# Autodesk Inventor assembly: Catapult Launcher
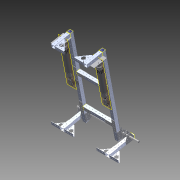
[picture p0: Inventor's stored thumbnail of the model, 180x180]
Saved by Autodesk Inventor 2014 (Build 180170000, 170)
## iProperties
Created: 2014-01-17
Part Number: Catapult Launcher
Document SubType Name: Assembly
Designer: Andrew Toennies
Mass: 1552.27 g
Surface Area: 5150.08 cm^2
Volume: 383.1 cm^3
Density: 4.05187 g/cm^3
Author: Andrew Toennies
## Documents named in this file (14)
- C:\Users\Andrew Toennies\Documents\GitHub\2014buildCAD\New Shooter\Catapult Launcher.iam
- C:\Users\Andrew Toennies\Documents\GitHub\2014buildCAD\New Shooter\Vex Pro 1x1 rectangular tubing 7 in length.ipt
- C:\Users\Andrew Toennies\Documents\GitHub\2014buildCAD\New Shooter\Vex Pro Side Bearing Gusset.ipt
- C:\Users\Andrew Toennies\Documents\GitHub\2014buildCAD\New Shooter\Vex Pro Corner Gusset.ipt
- C:\Users\Andrew Toennies\Documents\GitHub\2014buildCAD\New Shooter\Bearing ID 0.500 Hex OD 1.125.ipt
- C:\Users\Andrew Toennies\Documents\GitHub\2014buildCAD\New Shooter\Shaft (Steel 0.500 Hex).ipt
- C:\Users\Andrew Toennies\Documents\GitHub\2014buildCAD\New Shooter\Vex Pro 1x1 rectangular tubing 27 in length.ipt
- C:\Users\Andrew Toennies\Documents\GitHub\2014buildCAD\New Shooter\Vex Pro 1x1 rectangular tubing 3 in length.ipt
- C:\Users\Andrew Toennies\Documents\GitHub\2014buildCAD\New Shooter\Vex Pro 1x1 rectangular tubing 11 in length.ipt
- C:\Users\Andrew Toennies\Documents\GitHub\2014buildCAD\New Shooter\Vex Pro T gusset.ipt
- C:\Users\Andrew Toennies\Documents\GitHub\2014buildCAD\New Shooter\1.5 in bore 6 in stroke cylinder - BIMBA\176-DP(D-229)(F,D-231-1).iam
- C:\Users\Andrew Toennies\Documents\GitHub\2014buildCAD\New Shooter\Aluminum Plate (0.125).ipt
- C:\Users\Andrew Toennies\Documents\GitHub\2014buildCAD\New Shooter\1.5 in bore 6 in stroke cylinder - BIMBA\D-14826.ipt
- C:\Users\Andrew Toennies\Documents\GitHub\2014buildCAD\New Shooter\1.5 in bore 6 in stroke cylinder - BIMBA\D-9969.ipt
## Components (45 placed, 13 different names)
1. Shaft (Steel 0.500 Hex):1 — Mate:34, Mate:35, Flush:25
2. Vex Pro 1x1 rectangular tubing 3 in length:1 — Flush:13, Mate:118, Mate:119, Mate:120, Mate:123, Flush:19, Mate:160, Mate:212
3. Vex Pro 1x1 rectangular tubing 3 in length:2 — Mate:121, Flush:14, Mate:122, Flush:19, Mate:159
4. Vex Pro 1x1 rectangular tubing 11 in length:1 — Mate:140, Mate:141, Mate:142, Mate:143, Mate:146, Mate:147, Mate:148, Mate:149, Mate:191, Mate:193, Mate:194, Mate:196, Mate:197
5. Vex Pro 1x1 rectangular tubing 11 in length:2 — Mate:127, Mate:128, Mate:129, Mate:131, Mate:135, Mate:136, Mate:137, Mate:185
6. Vex Pro T gusset:1 — Mate:140, Mate:141, Mate:142, Mate:201, Mate:202
7. Vex Pro T gusset:2 — Mate:143, Mate:193, Mate:194
8. Vex Pro T gusset:3 — Mate:127, Mate:128, Mate:129, Mate:203, Mate:204, Mate:205
9. Vex Pro T gusset:4 — Mate:146, Mate:147, Mate:148
10. Vex Pro T gusset:5 — Mate:135, Mate:136, Mate:185
11. Vex Pro T gusset:6 — Mate:137, Mate:210, Mate:211
12. Vex Pro T gusset:7 — Mate:149, Mate:196, Mate:197
13. Vex Pro T gusset:8 — Mate:131, Mate:187, Mate:192
14. Aluminum Plate (0.125):1 — Mate:153, Mate:154, Mate:155, Mate:159, Flush:24
15. Aluminum Plate (0.125):2 — Mate:156, Mate:160, Mate:167, Mate:168, Flush:24
16. D-14826:1 — Mate:164, Mate:169, Mate:170, Mate:177, Mate:178
17. D-9969:1 — Mate:164, Mate:165, Mate:166, Mate:198, Mate:199, Mate:200
18. Vex Pro 1x1 rectangular tubing 27 in length:3 — Mate:198, Mate:199, Mate:200, Mate:201, Mate:202, Mate:203, Mate:204, Mate:205, Mate:206, Mate:207, Mate:208, Mate:209, Mate:213
19. Vex Pro 1x1 rectangular tubing 7 in length:1 — Flush:1, Flush:2, Mate:8, Mate:11, Mate:20, Mate:21, Mate:22, Mate:23, Mate:24, Mate:25, Mate:114, Mate:115, Mate:116, Mate:117, Mate:195
20. Vex Pro 1x1 rectangular tubing 7 in length:2 — Flush:1, Flush:2, Mate:3, Mate:5, Mate:14, Mate:15, Mate:16, Mate:17, Mate:18, Mate:19, Mate:110, Mate:111, Mate:112, Mate:113, Mate:123, Mate:188, Mate:195, Flush:25
21. Vex Pro Side Bearing Gusset:1 — Mate:3, Mate:26, Mate:27, Mate:110, Mate:111
22. Vex Pro Side Bearing Gusset:2 — Mate:5, Mate:28, Mate:29, Mate:112, Mate:113
23. Vex Pro Side Bearing Gusset:3 — Mate:11, Mate:32, Mate:33, Mate:116, Mate:117
24. Vex Pro Side Bearing Gusset:4 — Mate:8, Mate:30, Mate:31, Mate:114, Mate:115
25. Vex Pro Corner Gusset:1 — Mate:17, Mate:18, Mate:19, Flush:18
26. Vex Pro Corner Gusset:2 — Mate:14, Mate:15, Mate:16
27. Vex Pro Corner Gusset:3 — Mate:20, Mate:21, Mate:22
28. Vex Pro Corner Gusset:4 — Mate:23, Mate:24, Mate:25
29. Bearing ID 0.500 Hex OD 1.125:1 — Mate:28, Mate:29, Flush:3, Flush:5
30. Bearing ID 0.500 Hex OD 1.125:2 — Mate:26, Mate:27, Flush:3, Mate:34, Mate:35, Mate:44
31. Bearing ID 0.500 Hex OD 1.125:3 — Mate:30, Mate:31, Flush:4
32. Bearing ID 0.500 Hex OD 1.125:4 — Mate:32, Mate:33, Flush:4, Flush:5, Mate:69
33. Vex Pro Side Bearing Gusset:5 — Mate:57, Mate:58, Mate:180, Mate:181, Mate:189
34. Vex Pro Side Bearing Gusset:6 — Mate:55, Mate:56, Mate:208, Mate:209, Mate:213
35. Vex Pro Side Bearing Gusset:7 — Mate:51, Mate:52, Mate:206, Mate:207
36. Vex Pro Side Bearing Gusset:8 — Mate:44, Mate:53, Mate:54, Mate:179, Mate:182
37. Vex Pro 1x1 rectangular tubing 27 in length:2 — Mate:177, Mate:178, Mate:179, Mate:180, Mate:181, Mate:182, Mate:187, Mate:188, Mate:189, Mate:191, Mate:192, Mate:210, Mate:211, Mate:212
38. Bearing ID 0.500 Hex OD 1.125:5 — Mate:57, Mate:58, Mate:80
39. Bearing ID 0.500 Hex OD 1.125:6 — Mate:53, Mate:54, Mate:80
40. Bearing ID 0.500 Hex OD 1.125:7 — Mate:51, Mate:52, Mate:68, Mate:69
41. Bearing ID 0.500 Hex OD 1.125:8 — Mate:55, Mate:56, Mate:68
42. Vex Pro Corner Gusset:8 — Flush:13, Mate:118, Mate:119, Mate:120, Flush:17, Flush:18
43. Vex Pro Corner Gusset:6 — Mate:121, Flush:14, Mate:122, Flush:17
44. 176-DP(D-229)(F,D-231-1):1 [sub-assembly] — Mate:153, Mate:154, Mate:155, Mate:165, Mate:166, Mate:171
45. 176-DP(D-229)(F,D-231-1):2 [sub-assembly] — Mate:156, Mate:167, Mate:168, Mate:169, Mate:170, Mate:171
## Relationships (126: Mate 114, Flush 12)
- Flush:1: Vex Pro 1x1 rectangular tubing 7 in length:1 ↔ Vex Pro 1x1 rectangular tubing 7 in length:2
- Flush:2: Vex Pro 1x1 rectangular tubing 7 in length:1 ↔ Vex Pro 1x1 rectangular tubing 7 in length:2
- Mate:3: Vex Pro 1x1 rectangular tubing 7 in length:2 ↔ Vex Pro Side Bearing Gusset:1
- Mate:5: Vex Pro 1x1 rectangular tubing 7 in length:2 ↔ Vex Pro Side Bearing Gusset:2
- Mate:8: Vex Pro 1x1 rectangular tubing 7 in length:1 ↔ Vex Pro Side Bearing Gusset:4
- Mate:11: Vex Pro 1x1 rectangular tubing 7 in length:1 ↔ Vex Pro Side Bearing Gusset:3
- Mate:14: Vex Pro 1x1 rectangular tubing 7 in length:2 ↔ Vex Pro Corner Gusset:2
- Mate:15: Vex Pro 1x1 rectangular tubing 7 in length:2 ↔ Vex Pro Corner Gusset:2
- Mate:16: Vex Pro 1x1 rectangular tubing 7 in length:2 ↔ Vex Pro Corner Gusset:2
- Mate:17: Vex Pro 1x1 rectangular tubing 7 in length:2 ↔ Vex Pro Corner Gusset:1
- Mate:18: Vex Pro 1x1 rectangular tubing 7 in length:2 ↔ Vex Pro Corner Gusset:1
- Mate:19: Vex Pro 1x1 rectangular tubing 7 in length:2 ↔ Vex Pro Corner Gusset:1
- Mate:20: Vex Pro 1x1 rectangular tubing 7 in length:1 ↔ Vex Pro Corner Gusset:3
- Mate:21: Vex Pro 1x1 rectangular tubing 7 in length:1 ↔ Vex Pro Corner Gusset:3
- Mate:22: Vex Pro 1x1 rectangular tubing 7 in length:1 ↔ Vex Pro Corner Gusset:3
- Mate:23: Vex Pro 1x1 rectangular tubing 7 in length:1 ↔ Vex Pro Corner Gusset:4
- Mate:24: Vex Pro 1x1 rectangular tubing 7 in length:1 ↔ Vex Pro Corner Gusset:4
- Mate:25: Vex Pro 1x1 rectangular tubing 7 in length:1 ↔ Vex Pro Corner Gusset:4
- Mate:26: Vex Pro Side Bearing Gusset:1 ↔ Bearing ID 0.500 Hex OD 1.125:2
- Mate:27: Vex Pro Side Bearing Gusset:1 ↔ Bearing ID 0.500 Hex OD 1.125:2
- Mate:28: Vex Pro Side Bearing Gusset:2 ↔ Bearing ID 0.500 Hex OD 1.125:1
- Mate:29: Vex Pro Side Bearing Gusset:2 ↔ Bearing ID 0.500 Hex OD 1.125:1
- Flush:3: Bearing ID 0.500 Hex OD 1.125:1 ↔ Bearing ID 0.500 Hex OD 1.125:2
- Mate:30: Vex Pro Side Bearing Gusset:4 ↔ Bearing ID 0.500 Hex OD 1.125:3
- Mate:31: Vex Pro Side Bearing Gusset:4 ↔ Bearing ID 0.500 Hex OD 1.125:3
- Mate:32: Vex Pro Side Bearing Gusset:3 ↔ Bearing ID 0.500 Hex OD 1.125:4
- Mate:33: Vex Pro Side Bearing Gusset:3 ↔ Bearing ID 0.500 Hex OD 1.125:4
- Flush:4: Bearing ID 0.500 Hex OD 1.125:3 ↔ Bearing ID 0.500 Hex OD 1.125:4
- Flush:5: Bearing ID 0.500 Hex OD 1.125:1 ↔ Bearing ID 0.500 Hex OD 1.125:4
- Mate:34: Shaft (Steel 0.500 Hex):1 ↔ Bearing ID 0.500 Hex OD 1.125:2
- Mate:35: Shaft (Steel 0.500 Hex):1 ↔ Bearing ID 0.500 Hex OD 1.125:2
- Mate:44: Bearing ID 0.500 Hex OD 1.125:2 ↔ Vex Pro Side Bearing Gusset:8
- Mate:51: Vex Pro Side Bearing Gusset:7 ↔ Bearing ID 0.500 Hex OD 1.125:7
- Mate:52: Vex Pro Side Bearing Gusset:7 ↔ Bearing ID 0.500 Hex OD 1.125:7
- Mate:53: Vex Pro Side Bearing Gusset:8 ↔ Bearing ID 0.500 Hex OD 1.125:6
- Mate:54: Vex Pro Side Bearing Gusset:8 ↔ Bearing ID 0.500 Hex OD 1.125:6
- Mate:55: Vex Pro Side Bearing Gusset:6 ↔ Bearing ID 0.500 Hex OD 1.125:8
- Mate:56: Vex Pro Side Bearing Gusset:6 ↔ Bearing ID 0.500 Hex OD 1.125:8
- Mate:57: Vex Pro Side Bearing Gusset:5 ↔ Bearing ID 0.500 Hex OD 1.125:5
- Mate:58: Vex Pro Side Bearing Gusset:5 ↔ Bearing ID 0.500 Hex OD 1.125:5
- Mate:68: Bearing ID 0.500 Hex OD 1.125:7 ↔ Bearing ID 0.500 Hex OD 1.125:8
- Mate:69: Bearing ID 0.500 Hex OD 1.125:4 ↔ Bearing ID 0.500 Hex OD 1.125:7
- Mate:80: Bearing ID 0.500 Hex OD 1.125:5 ↔ Bearing ID 0.500 Hex OD 1.125:6
- Mate:110: Vex Pro 1x1 rectangular tubing 7 in length:2 ↔ Vex Pro Side Bearing Gusset:1
- Mate:111: Vex Pro 1x1 rectangular tubing 7 in length:2 ↔ Vex Pro Side Bearing Gusset:1
- Mate:112: Vex Pro 1x1 rectangular tubing 7 in length:2 ↔ Vex Pro Side Bearing Gusset:2
- Mate:113: Vex Pro 1x1 rectangular tubing 7 in length:2 ↔ Vex Pro Side Bearing Gusset:2
- Mate:114: Vex Pro 1x1 rectangular tubing 7 in length:1 ↔ Vex Pro Side Bearing Gusset:4
- Mate:115: Vex Pro 1x1 rectangular tubing 7 in length:1 ↔ Vex Pro Side Bearing Gusset:4
- Mate:116: Vex Pro 1x1 rectangular tubing 7 in length:1 ↔ Vex Pro Side Bearing Gusset:3
- Mate:117: Vex Pro 1x1 rectangular tubing 7 in length:1 ↔ Vex Pro Side Bearing Gusset:3
- Flush:13: Vex Pro 1x1 rectangular tubing 3 in length:1 ↔ Vex Pro Corner Gusset:8
- Mate:118: Vex Pro 1x1 rectangular tubing 3 in length:1 ↔ Vex Pro Corner Gusset:8
- Mate:119: Vex Pro 1x1 rectangular tubing 3 in length:1 ↔ Vex Pro Corner Gusset:8
- Mate:120: Vex Pro 1x1 rectangular tubing 3 in length:1 ↔ Vex Pro Corner Gusset:8
- Mate:121: Vex Pro 1x1 rectangular tubing 3 in length:2 ↔ Vex Pro Corner Gusset:6
- Flush:14: Vex Pro 1x1 rectangular tubing 3 in length:2 ↔ Vex Pro Corner Gusset:6
- Mate:122: Vex Pro 1x1 rectangular tubing 3 in length:2 ↔ Vex Pro Corner Gusset:6
- Flush:17: Vex Pro Corner Gusset:8 ↔ Vex Pro Corner Gusset:6
- Flush:18: Vex Pro Corner Gusset:1 ↔ Vex Pro Corner Gusset:8
- Mate:123 (-685.8 mm): Vex Pro 1x1 rectangular tubing 3 in length:1 ↔ Vex Pro 1x1 rectangular tubing 7 in length:2
- Flush:19: Vex Pro 1x1 rectangular tubing 3 in length:1 ↔ Vex Pro 1x1 rectangular tubing 3 in length:2
- Mate:127: Vex Pro 1x1 rectangular tubing 11 in length:2 ↔ Vex Pro T gusset:3
- Mate:128: Vex Pro 1x1 rectangular tubing 11 in length:2 ↔ Vex Pro T gusset:3
- Mate:129: Vex Pro 1x1 rectangular tubing 11 in length:2 ↔ Vex Pro T gusset:3
- Mate:131: Vex Pro 1x1 rectangular tubing 11 in length:2 ↔ Vex Pro T gusset:8
- Mate:135: Vex Pro 1x1 rectangular tubing 11 in length:2 ↔ Vex Pro T gusset:5
- Mate:136: Vex Pro 1x1 rectangular tubing 11 in length:2 ↔ Vex Pro T gusset:5
- Mate:137: Vex Pro 1x1 rectangular tubing 11 in length:2 ↔ Vex Pro T gusset:6
- Mate:140: Vex Pro 1x1 rectangular tubing 11 in length:1 ↔ Vex Pro T gusset:1
- Mate:141: Vex Pro 1x1 rectangular tubing 11 in length:1 ↔ Vex Pro T gusset:1
- Mate:142: Vex Pro 1x1 rectangular tubing 11 in length:1 ↔ Vex Pro T gusset:1
- Mate:143: Vex Pro 1x1 rectangular tubing 11 in length:1 ↔ Vex Pro T gusset:2
- Mate:146: Vex Pro 1x1 rectangular tubing 11 in length:1 ↔ Vex Pro T gusset:4
- Mate:147: Vex Pro 1x1 rectangular tubing 11 in length:1 ↔ Vex Pro T gusset:4
- Mate:148: Vex Pro 1x1 rectangular tubing 11 in length:1 ↔ Vex Pro T gusset:4
- Mate:149: Vex Pro 1x1 rectangular tubing 11 in length:1 ↔ Vex Pro T gusset:7
- Mate:153: Aluminum Plate (0.125):1 ↔ 176-DP(D-229)(F,D-231-1):1
- Mate:154: Aluminum Plate (0.125):1 ↔ 176-DP(D-229)(F,D-231-1):1
- Mate:155: Aluminum Plate (0.125):1 ↔ 176-DP(D-229)(F,D-231-1):1
- Mate:156: Aluminum Plate (0.125):2 ↔ 176-DP(D-229)(F,D-231-1):2
- Mate:159: Vex Pro 1x1 rectangular tubing 3 in length:2 ↔ Aluminum Plate (0.125):1
- Mate:160: Vex Pro 1x1 rectangular tubing 3 in length:1 ↔ Aluminum Plate (0.125):2
- Mate:164: D-14826:1 ↔ D-9969:1
- Mate:165: D-9969:1 ↔ 176-DP(D-229)(F,D-231-1):1
- Mate:166 (3.2131 mm): D-9969:1 ↔ 176-DP(D-229)(F,D-231-1):1
- Mate:167: Aluminum Plate (0.125):2 ↔ 176-DP(D-229)(F,D-231-1):2
- Mate:168: Aluminum Plate (0.125):2 ↔ 176-DP(D-229)(F,D-231-1):2
- Mate:169: D-14826:1 ↔ 176-DP(D-229)(F,D-231-1):2
- Mate:170 (3.2131 mm): D-14826:1 ↔ 176-DP(D-229)(F,D-231-1):2
- Mate:171: 176-DP(D-229)(F,D-231-1):1 ↔ 176-DP(D-229)(F,D-231-1):2
- Flush:24: Aluminum Plate (0.125):1 ↔ Aluminum Plate (0.125):2
- Mate:177: D-14826:1 ↔ Vex Pro 1x1 rectangular tubing 27 in length:2
- Mate:178: D-14826:1 ↔ Vex Pro 1x1 rectangular tubing 27 in length:2
- Mate:179: Vex Pro Side Bearing Gusset:8 ↔ Vex Pro 1x1 rectangular tubing 27 in length:2
- Mate:180: Vex Pro Side Bearing Gusset:5 ↔ Vex Pro 1x1 rectangular tubing 27 in length:2
- Mate:181: Vex Pro Side Bearing Gusset:5 ↔ Vex Pro 1x1 rectangular tubing 27 in length:2
- Mate:182: Vex Pro Side Bearing Gusset:8 ↔ Vex Pro 1x1 rectangular tubing 27 in length:2
- Mate:185: Vex Pro 1x1 rectangular tubing 11 in length:2 ↔ Vex Pro T gusset:5
- Mate:187: Vex Pro T gusset:8 ↔ Vex Pro 1x1 rectangular tubing 27 in length:2
- Mate:188 (25.4 mm): Vex Pro 1x1 rectangular tubing 7 in length:2 ↔ Vex Pro 1x1 rectangular tubing 27 in length:2
- Mate:189: Vex Pro Side Bearing Gusset:5 ↔ Vex Pro 1x1 rectangular tubing 27 in length:2
- Mate:191: Vex Pro 1x1 rectangular tubing 11 in length:1 ↔ Vex Pro 1x1 rectangular tubing 27 in length:2
- Mate:192: Vex Pro T gusset:8 ↔ Vex Pro 1x1 rectangular tubing 27 in length:2
- Mate:193: Vex Pro 1x1 rectangular tubing 11 in length:1 ↔ Vex Pro T gusset:2
- Mate:194: Vex Pro 1x1 rectangular tubing 11 in length:1 ↔ Vex Pro T gusset:2
- Mate:195 (330.2 mm): Vex Pro 1x1 rectangular tubing 7 in length:1 ↔ Vex Pro 1x1 rectangular tubing 7 in length:2
- Flush:25 (-25.4 mm): Shaft (Steel 0.500 Hex):1 ↔ Vex Pro 1x1 rectangular tubing 7 in length:2
- Mate:196: Vex Pro 1x1 rectangular tubing 11 in length:1 ↔ Vex Pro T gusset:7
- Mate:197: Vex Pro 1x1 rectangular tubing 11 in length:1 ↔ Vex Pro T gusset:7
- Mate:198: D-9969:1 ↔ Vex Pro 1x1 rectangular tubing 27 in length:3
- Mate:199: D-9969:1 ↔ Vex Pro 1x1 rectangular tubing 27 in length:3
- Mate:200: D-9969:1 ↔ Vex Pro 1x1 rectangular tubing 27 in length:3
- Mate:201: Vex Pro T gusset:1 ↔ Vex Pro 1x1 rectangular tubing 27 in length:3
- Mate:202: Vex Pro T gusset:1 ↔ Vex Pro 1x1 rectangular tubing 27 in length:3
- Mate:203: Vex Pro T gusset:3 ↔ Vex Pro 1x1 rectangular tubing 27 in length:3
- Mate:204: Vex Pro T gusset:3 ↔ Vex Pro 1x1 rectangular tubing 27 in length:3
- Mate:205: Vex Pro T gusset:3 ↔ Vex Pro 1x1 rectangular tubing 27 in length:3
- Mate:206: Vex Pro 1x1 rectangular tubing 27 in length:3 ↔ Vex Pro Side Bearing Gusset:7
- Mate:207: Vex Pro 1x1 rectangular tubing 27 in length:3 ↔ Vex Pro Side Bearing Gusset:7
- Mate:208: Vex Pro 1x1 rectangular tubing 27 in length:3 ↔ Vex Pro Side Bearing Gusset:6
- Mate:209: Vex Pro 1x1 rectangular tubing 27 in length:3 ↔ Vex Pro Side Bearing Gusset:6
- Mate:210: Vex Pro T gusset:6 ↔ Vex Pro 1x1 rectangular tubing 27 in length:2
- Mate:211: Vex Pro T gusset:6 ↔ Vex Pro 1x1 rectangular tubing 27 in length:2
- Mate:212: Vex Pro 1x1 rectangular tubing 3 in length:1 ↔ Vex Pro 1x1 rectangular tubing 27 in length:2
- Mate:213: Vex Pro 1x1 rectangular tubing 27 in length:3 ↔ Vex Pro Side Bearing Gusset:6
